# Autodesk Inventor assembly: Aero_assembly
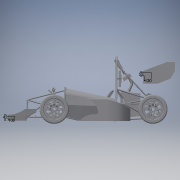
[picture p0: Inventor's stored thumbnail of the model, 180x180]
Saved by Autodesk Inventor 2018.2 (Build 222227000, 227)
## iProperties
Created: 2018-03-12
Part Number: Aero_assembly
Material: 一般
Document SubType Name: Assembly
Designer: ku_sk
Author: ku_sk
## Documents named in this file (4)
- C:\Users\ku_sk\Documents\Inventor\Aero\KS-15\Aero_assembly.iam
- C:\Users\ku_sk\Documents\Inventor\Aero\KS-15\body\2018 body assembly.iam
- C:\Users\ku_sk\Documents\Inventor\Aero\KS-15\Fr.wing\Fr.wing_assy.iam
- C:\Users\ku_sk\Documents\Inventor\Aero\KS-15\Rr.wing\Rr.wing_assy.iam
## Components (3 placed, 3 different names)
1. 2018 body assembly:1 [sub-assembly] — メイト:1, メイト:2, メイト:3, フラッシュ:5, メイト:8
2. Fr.wing_assy:1 [sub-assembly] — フラッシュ:1, フラッシュ:5, メイト:8
3. Rr.wing_assy:1 [sub-assembly] — フラッシュ:6, フラッシュ:7, メイト:7
## Relationships (9: Mate 5, Flush 4)
- メイト:1 [Mate]: 2018 body assembly:1
- メイト:2 [Mate]: 2018 body assembly:1
- メイト:3 [Mate]: 2018 body assembly:1
- フラッシュ:1 [Flush]: Fr.wing_assy:1
- フラッシュ:5 [Flush] (6 mm): 2018 body assembly:1 ↔ Fr.wing_assy:1
- フラッシュ:6 [Flush]: Rr.wing_assy:1
- フラッシュ:7 [Flush] (460 mm): Rr.wing_assy:1
- メイト:7 [Mate] (700 mm): Rr.wing_assy:1
- メイト:8 [Mate] (310 mm): 2018 body assembly:1 ↔ Fr.wing_assy:1
